# Autodesk Inventor assembly: Assembly2
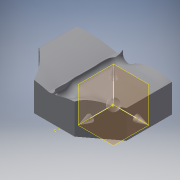
[picture p0: Inventor's stored thumbnail of the model, 180x180]
Saved by Autodesk Inventor 2018.1 (Build 221171000, 171)
## iProperties
Created: 2017-10-26
Part Number: Assembly2
Material: 一般
Document SubType Name: Assembly
Designer: KITformula
Author: KITformula
## Documents named in this file (3)
- C:\Users\formula\Dropbox\ishizaka\side1\Assembly2.iam
- C:\Users\formula\Dropbox\ishizaka\side1\part\ishispe.ipt
- C:\Users\formula\Dropbox\ishizaka\side1\part\ishispe_MIR.ipt
## Components (2 placed, 2 different names)
1. ishispe:1 — フラッシュ:2, フラッシュ:3, フラッシュ:4
2. ishispe_MIR:1 — フラッシュ:5, メイト:2, メイト:3
## Relationships (6: Flush 4, Mate 2)
- フラッシュ:2 [Flush]: ishispe:1
- フラッシュ:3 [Flush]: ishispe:1
- フラッシュ:4 [Flush]: ishispe:1
- フラッシュ:5 [Flush]: ishispe_MIR:1
- メイト:2 [Mate]: ishispe_MIR:1
- メイト:3 [Mate]: ishispe_MIR:1
